# Autodesk Inventor assembly: Assembly1
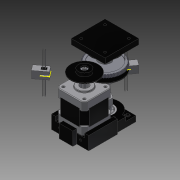
[picture p0: Inventor's stored thumbnail of the model, 180x180]
Saved by Autodesk Inventor 2015 (Build 190159000, 159)
## iProperties
Created: 2017-01-13
Part Number: Assembly1
Document SubType Name: Assembly
Designer: 1esh9
Author: 1esh9
## Documents named in this file (15)
- C:\Users\Ernest\Documents\Capstone-Project\doc\CAD\EndEffectorBase\Assembly1.iam
- C:\Users\Ernest\Documents\Capstone-Project\doc\CAD\EndEffectorBase\EEThreadedRod.ipt
- C:\Users\Ernest\Documents\Capstone-Project\doc\CAD\EndEffectorBase\BallBearingCone.ipt
- C:\Users\Ernest\Documents\Capstone-Project\doc\CAD\EndEffectorBase\BallBearingCup.ipt
- C:\Users\Ernest\Documents\Capstone-Project\doc\CAD\EndEffectorBase\BallBearing.ipt
- C:\Users\Ernest\Documents\Capstone-Project\doc\CAD\EndEffectorBase\BallBearingConeLockNut.ipt
- C:\Users\Ernest\Documents\Capstone-Project\doc\CAD\EndEffectorBase\BallBearingCupMount.ipt
- C:\Users\Ernest\Documents\Capstone-Project\doc\CAD\EndEffectorBase\EEThreadedRodNut.ipt
- C:\Users\Ernest\Documents\Capstone-Project\doc\CAD\Gears\Spur Gears1.iam
- C:\Users\Ernest\Documents\Capstone-Project\doc\CAD\Stepper Motor\NEMA-17\NEMA 17.iam
- C:\Users\Ernest\Documents\Capstone-Project\doc\CAD\EndEffectorBase\BallBearingCupMountBottom.ipt
- C:\Users\Ernest\Documents\Capstone-Project\doc\CAD\EndEffectorBase\SmallPositionDisk.ipt
- C:\Users\Ernest\Documents\Capstone-Project\doc\CAD\EndEffectorBase\BigPositionDisk.ipt
- C:\Users\Ernest\Documents\Capstone-Project\doc\CAD\Sensors\LineSensor.ipt
- C:\Users\Ernest\Documents\Capstone-Project\doc\CAD\Sensors\LinesensorHolder.ipt
## Components (23 placed, 14 different names)
1. EEThreadedRod:1 — Mate:1, Mate:2, Mate:3, Mate:4, Mate:5, Mate:6, Mate:7, Mate:10, Mate:11, Mate:18, Mate:19, Mate:20, Flush:1, Mate:22, Mate:27
2. BallBearingCone:1 — Mate:2, Mate:8, Flush:1
3. BallBearingCone:2 — Mate:3, Mate:9
4. BallBearingCup:1 — Mate:4, Tangent:1, Mate:8, Mate:16, Mate:17
5. BallBearingCup:2 — Mate:5, Tangent:2, Mate:9, Mate:23
6. BallBearing:1 — Mate:6, Tangent:1
7. BallBearing:2 — Mate:7, Tangent:2
8. BallBearingConeLockNut:1 — Mate:10
9. BallBearingConeLockNut:2 — Mate:11
10. BallBearingCupMount:2 — Mate:16, Mate:17, Angle:3
11. EEThreadedRodNut:1 — Mate:18
12. EEThreadedRodNut:2 — Mate:19
13. Spur Gears:1 [sub-assembly] — Mate:20, Mate:21, Mate:25, Mate:26
14. NEMA 17:1 [sub-assembly] — Mate:21, Flush:2, Mate:24
15. BallBearingCupMountBottom:1 — Mate:22, Mate:23, Flush:2, Mate:24, Angle:2, Angle:3
16. SmallPositionDisk:1 — Mate:25, Mate:26, Mate:33
17. BigPositionDisk:1 — Mate:27, Flush:11, Flush:12, Mate:32
18. LineSensor:1 — Flush:3, Flush:4, Mate:30, Mate:31, Flush:9
19. LineSensor:2 — Flush:3, Flush:4, Flush:10, Flush:11, Flush:12
20. LineSensor:3 — Flush:5, Flush:6, Mate:28, Mate:29, Flush:7
21. LineSensor:4 — Flush:5, Flush:6, Flush:8, Mate:33
22. LinesensorHolder:1 — Mate:28, Mate:29, Flush:7, Flush:8
23. LinesensorHolder:2 — Mate:30, Mate:31, Flush:9, Flush:10, Mate:32
## Relationships (45: Mate 29, Flush 12, Tangent 2, Angle 2)
- Mate:1: EEThreadedRod:1
- Mate:2: EEThreadedRod:1 ↔ BallBearingCone:1
- Mate:3: EEThreadedRod:1 ↔ BallBearingCone:2
- Mate:4: EEThreadedRod:1 ↔ BallBearingCup:1
- Mate:5: EEThreadedRod:1 ↔ BallBearingCup:2
- Mate:6: EEThreadedRod:1 ↔ BallBearing:1
- Mate:7: EEThreadedRod:1 ↔ BallBearing:2
- Tangent:1: BallBearingCup:1 ↔ BallBearing:1
- Mate:8 (-16.3 mm): BallBearingCone:1 ↔ BallBearingCup:1
- Tangent:2: BallBearingCup:2 ↔ BallBearing:2
- Mate:9 (-16.3 mm): BallBearingCone:2 ↔ BallBearingCup:2
- Mate:10: EEThreadedRod:1 ↔ BallBearingConeLockNut:1
- Mate:11: EEThreadedRod:1 ↔ BallBearingConeLockNut:2
- Mate:16: BallBearingCup:1 ↔ BallBearingCupMount:2
- Mate:17: BallBearingCup:1 ↔ BallBearingCupMount:2
- Mate:18: EEThreadedRod:1 ↔ EEThreadedRodNut:1
- Mate:19: EEThreadedRod:1 ↔ EEThreadedRodNut:2
- Mate:20: EEThreadedRod:1 ↔ Spur Gears:1
- Mate:21: Spur Gears:1 ↔ NEMA 17:1
- Flush:1: EEThreadedRod:1 ↔ BallBearingCone:1
- Mate:22: EEThreadedRod:1 ↔ BallBearingCupMountBottom:1
- Mate:23: BallBearingCup:2 ↔ BallBearingCupMountBottom:1
- Flush:2: NEMA 17:1 ↔ BallBearingCupMountBottom:1
- Mate:24: NEMA 17:1 ↔ BallBearingCupMountBottom:1
- Mate:25: Spur Gears:1 ↔ SmallPositionDisk:1
- Mate:26: Spur Gears:1 ↔ SmallPositionDisk:1
- Mate:27: EEThreadedRod:1 ↔ BigPositionDisk:1
- Flush:3: LineSensor:1 ↔ LineSensor:2
- Flush:4: LineSensor:1 ↔ LineSensor:2
- Flush:5: LineSensor:3 ↔ LineSensor:4
- Flush:6: LineSensor:3 ↔ LineSensor:4
- Angle:2 (0 deg): BallBearingCupMountBottom:1
- Mate:28 (0.2 mm): LineSensor:3 ↔ LinesensorHolder:1
- Mate:29 (0.2 mm): LineSensor:3 ↔ LinesensorHolder:1
- Flush:7: LineSensor:3 ↔ LinesensorHolder:1
- Flush:8: LineSensor:4 ↔ LinesensorHolder:1
- Mate:30 (0.2 mm): LineSensor:1 ↔ LinesensorHolder:2
- Mate:31 (0.2 mm): LineSensor:1 ↔ LinesensorHolder:2
- Flush:9: LineSensor:1 ↔ LinesensorHolder:2
- Flush:10: LineSensor:2 ↔ LinesensorHolder:2
- Angle:3 (0 deg): BallBearingCupMount:2 ↔ BallBearingCupMountBottom:1
- Flush:11 (-0.7 mm): BigPositionDisk:1 ↔ LineSensor:2
- Flush:12 (0.2 mm): BigPositionDisk:1 ↔ LineSensor:2
- Mate:32 (0.201 mm): BigPositionDisk:1 ↔ LinesensorHolder:2
- Mate:33 (0.2 mm): SmallPositionDisk:1 ↔ LineSensor:4
